# Autodesk Inventor assembly: FE-00004-02
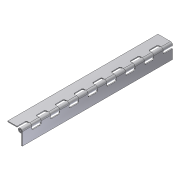
[picture p0: Inventor's stored thumbnail of the model, 180x180]
Saved by Autodesk Inventor 2012 (Build 160160000, 160)
## iProperties
Created: 2008-05-29
Part Number: FE-00004-02
Document SubType Name: Assembly
Designer: narosenberg
Description: Hinge, End Shelf
Author: narosenberg
## Documents named in this file (3)
- C:\Data Folder\FRC 2012 Field\Components\FE-00004-02.iam
- C:\Data Folder\FRC 2012 Field\Components\FE-00004-02A.ipt
- C:\Data Folder\FRC 2012 Field\Components\FE-00004-02C.ipt
## Components (3 placed, 2 different names)
1. FE-00004-02A:1 — Insert:1, Insert:2, Angle:1
2. FE-00004-02A:2 — Insert:1, Angle:1
3. FE-00004-02C:1 — Insert:2
## Relationships (3: Insert 2, Angle 1)
- Insert:1: FE-00004-02A:1 ↔ FE-00004-02A:2
- Insert:2: FE-00004-02A:1 ↔ FE-00004-02C:1
- Angle:1 (90 deg): FE-00004-02A:1 ↔ FE-00004-02A:2
